# Autodesk Inventor assembly: McCrea_BODY_walle
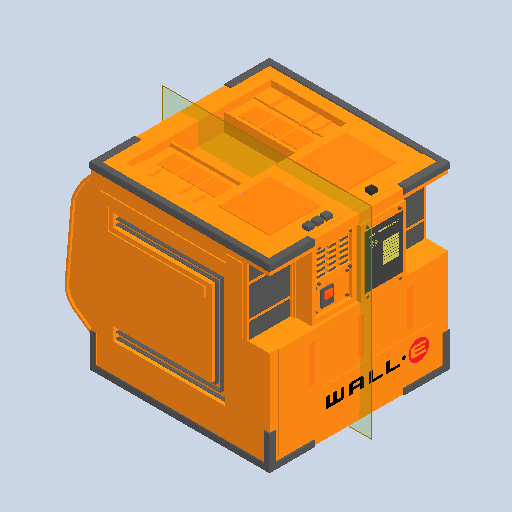
[picture p0: Inventor's stored thumbnail of the model, 512x512]
Saved by Autodesk Inventor 2022 (Build 260153000, 153)
## iProperties
Created: 2022-01-08
Part Number: McCrea_BODY_walle
Document SubType Name: Assembly
Designer: Lukas
Author: Lukas
## Documents named in this file (4)
- C:\Users\Lukas\Desktop\ard\3D\Walle\FINAL\lukas\McCrea_BODY_walle.iam
- C:\Users\Lukas\Desktop\ard\3D\Walle\FINAL\lukas\McCrea_body_walle.ipt
- C:\Users\Lukas\Desktop\ard\3D\Walle\FINAL\lukas\McCrea_bodyzadokfinal_walle.iam
- McCrea_bodyzadokfinal_walle.ipt
## Components (2 placed, 2 different names)
1. McCrea_body_walle:1 — Insert:1, Flush:1
2. McCrea_bodyzadokfinal_walle:1 [sub-assembly] — Insert:1
## Relationships (2: Insert 1, Flush 1)
- Insert:1: McCrea_body_walle:1 ↔ McCrea_bodyzadokfinal_walle:1
- Flush:1 (-40 mm): McCrea_body_walle:1
